# Autodesk Inventor assembly: Assembly2
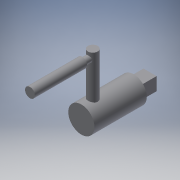
[picture p0: Inventor's stored thumbnail of the model, 180x180]
Saved by Autodesk Inventor 2019 (Build 230136000, 136)
## iProperties
Created: 2019-05-03
Part Number: Assembly2
Document SubType Name: Assembly
Designer: samson.bailor
Author: samson.bailor
## Documents named in this file (4)
- S:\Modern Technology Academy\Bogdziewicz\Student Drop Box\1-Collaboration\47-EDD-2019\Trotline\trotline-reel\src\inventor\Assembly2.iam
- S:\Modern Technology Academy\Bogdziewicz\Student Drop Box\1-Collaboration\47-EDD-2019\Trotline\trotline-reel\src\inventor\CrankP1_SBail.ipt
- S:\Modern Technology Academy\Bogdziewicz\Student Drop Box\1-Collaboration\47-EDD-2019\Trotline\trotline-reel\src\inventor\CrankP2_SBail.ipt
- S:\Modern Technology Academy\Bogdziewicz\Student Drop Box\1-Collaboration\47-EDD-2019\Trotline\trotline-reel\src\inventor\CrankHandle_SBail.ipt
## Components (3 placed, 3 different names)
1. CrankP1_SBail:1 — Insert:1
2. CrankP2_SBail:1 — Insert:1, Mate:1
3. CrankHandle_SBail:1 — Mate:1
## Relationships (2: Insert 1, Mate 1)
- Insert:1: CrankP1_SBail:1 ↔ CrankP2_SBail:1
- Mate:1: CrankP2_SBail:1 ↔ CrankHandle_SBail:1
